# Autodesk Inventor assembly: ShoulderBearingUnitBasis
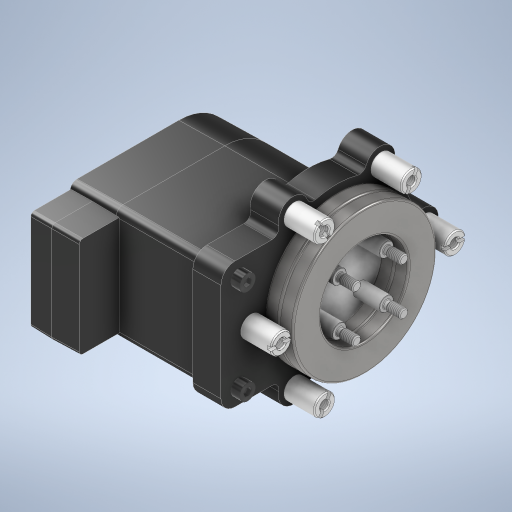
[picture p0: Inventor's stored thumbnail of the model, 512x512]
Saved by Autodesk Inventor 2024.2 (Build 282272000, 272)
## iProperties
Created: 2024-01-04
Part Number: ShoulderBearingUnitBasis
Document SubType Name: Assembly
Designer: Masato Kubotera
Mass: 101.427 g
Surface Area: 162.729 cm^2
Volume: 22.4446 cm^3
Density: 4.51898 g/cm^3
Author: Masato Kubotera
## Documents named in this file (10)
- C:\Users\masato\OneDrive - Chiba Institute of Technology\CIT Brains\RoboCup2024\Mechanic\SUSTAINA-OP2-DEV - 作業\NativeFiles\Boby\UpperLimb\Shoulders\ShoulderBearingUnitBasis.iam
- C:\Users\masato\OneDrive - Chiba Institute of Technology\CIT Brains\RoboCup2024\Mechanic\SUSTAINA-OP2-DEV - 作業\NativeFiles\Boby\COTS\Bearings\RB2508UUC0.ipt
- C:\Users\masato\OneDrive - Chiba Institute of Technology\CIT Brains\RoboCup2024\Mechanic\SUSTAINA-OP2-DEV - 作業\NativeFiles\Boby\CommonDesignedComponents\CrossRollerBearingUnit\CrossRollerBearingInnerFlange.ipt
- C:\Users\masato\OneDrive - Chiba Institute of Technology\CIT Brains\RoboCup2024\Mechanic\SUSTAINA-OP2-DEV - 作業\NativeFiles\Boby\UpperLimb\Shoulders\ShoulderBearingOuterFlange.ipt
- C:\Users\masato\OneDrive - Chiba Institute of Technology\CIT Brains\RoboCup2024\Mechanic\SUSTAINA-OP2-DEV - 作業\NativeFiles\Boby\COTS\Spacers\ARU-309S.ipt
- C:\Users\masato\OneDrive - Chiba Institute of Technology\CIT Brains\RoboCup2024\Mechanic\SUSTAINA-OP2-DEV - 作業\NativeFiles\Boby\COTS\Spacers\BRU-309S.ipt
- C:\Users\masato\OneDrive - Chiba Institute of Technology\CIT Brains\RoboCup2024\Mechanic\SUSTAINA-OP2-DEV - 作業\NativeFiles\Boby\COTS\Screws\ScrewsWithShoulder\LMSBP4-10.ipt
- C:\Users\masato\OneDrive - Chiba Institute of Technology\CIT Brains\RoboCup2024\Mechanic\SUSTAINA-OP2-DEV - 作業\NativeFiles\Boby\COTS\Screws\CapScrew\UC-0306.ipt
- C:\Users\masato\OneDrive - Chiba Institute of Technology\CIT Brains\RoboCup2024\Mechanic\SUSTAINA-OP2-DEV - 作業\NativeFiles\Boby\COTS\Screws\CapScrew\FC-2615EB.ipt
- C:\Users\masato\OneDrive - Chiba Institute of Technology\CIT Brains\RoboCup2024\Mechanic\SUSTAINA-OP2-DEV - 作業\NativeFiles\Boby\COTS\Actuators\PMX-SCR-9204HV.ipt
## Components (17 placed, 9 different names)
1. Shoulder_CrossRollerBearingOuterFlange:1 — Insert:12, Insert:13, Insert:14, Insert:15, Insert:17, Insert:18, Insert:19, Insert:20, Mate:1, Mate:2, Mate:3, Mate:4
2. CrossRollerBearingInnerFlange:1 — Insert:7, Angle:4, Insert:16
3. PMX-SCR-9204HV:1 — Insert:17, Insert:18
4. FC-2615EB:1 — Insert:19
5. FC-2615EB:2 — Insert:20
6. UC-0306:1 — Insert:15
7. ARU-309S:1 — Insert:14, Angle:10
8. RB2508UUC0:1 — Insert:7, Insert:12
9. BRU-309S:1 — Insert:13, Angle:11
10. BRU-309S:2
11. BRU-309S:3
12. BRU-309S:4
13. BRU-309S:5
14. LMSBP4-10:1 — Insert:16
15. LMSBP4-10:2
16. LMSBP4-10:3
17. LMSBP4-10:4
## Component patterns: (5 elements, first: BRU-309S:1), (4 elements, first: LMSBP4-10:1)
## Relationships (17: Insert 10, Mate 4, Angle 3)
- Insert:7: CrossRollerBearingInnerFlange:1 ↔ RB2508UUC0:1
- Angle:4 (0 deg): CrossRollerBearingInnerFlange:1
- Insert:12: Shoulder_CrossRollerBearingOuterFlange:1 ↔ RB2508UUC0:1
- Insert:13: Shoulder_CrossRollerBearingOuterFlange:1 ↔ BRU-309S:1
- Insert:14: Shoulder_CrossRollerBearingOuterFlange:1 ↔ ARU-309S:1
- Angle:10 (0 deg): ARU-309S:1
- Angle:11 (60 deg): BRU-309S:1
- Insert:15: Shoulder_CrossRollerBearingOuterFlange:1 ↔ UC-0306:1
- Insert:16: CrossRollerBearingInnerFlange:1 ↔ LMSBP4-10:1
- Insert:17: Shoulder_CrossRollerBearingOuterFlange:1 ↔ PMX-SCR-9204HV:1
- Insert:18: Shoulder_CrossRollerBearingOuterFlange:1 ↔ PMX-SCR-9204HV:1
- Insert:19: Shoulder_CrossRollerBearingOuterFlange:1 ↔ FC-2615EB:1
- Insert:20: Shoulder_CrossRollerBearingOuterFlange:1 ↔ FC-2615EB:2
- Mate:1: Shoulder_CrossRollerBearingOuterFlange:1
- Mate:2: Shoulder_CrossRollerBearingOuterFlange:1
- Mate:3: Shoulder_CrossRollerBearingOuterFlange:1
- Mate:4: Shoulder_CrossRollerBearingOuterFlange:1
